# Autodesk Inventor assembly: cosel-psu-din-clip
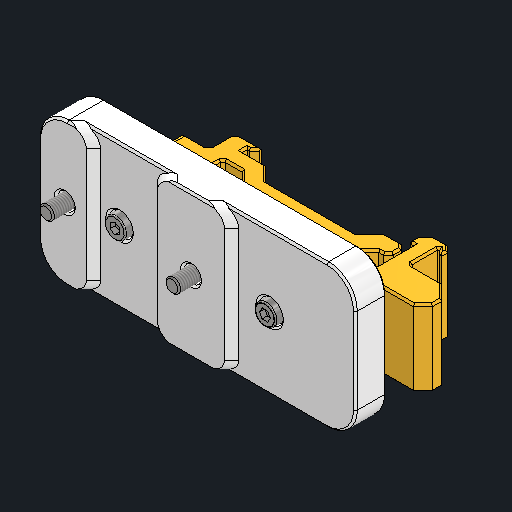
[picture p0: Inventor's stored thumbnail of the model, 512x512]
Saved by Autodesk Inventor 2026 (Build 300175050, 175E)
## iProperties
Created: 2026-03-04
Part Number: cosel-psu-din-clip
Document SubType Name: Assembly
Designer: kuzmin
Author: kuzmin
## Documents named in this file (5)
- C:\Users\queez\Dropbox\Drawings\PIHTI\ElectronicsBox\Win-GPIO-Box\cosel-psu-din-clip.iam
- C:\Users\queez\Dropbox\Drawings\PIHTI\ElectronicsBox\Win-GPIO-Box\Wide Din Clip.ipt
- C:\Users\queez\Dropbox\Drawings\PIHTI\ElectronicsBox\Win-GPIO-Box\cosel-psu-bracket.ipt
- C:\Users\queez\Dropbox\Drawings\PIHTI\ContentCenter\Fastners\M2.5x10-SHCS.ipt
- C:\Users\queez\Dropbox\Drawings\PIHTI\ContentCenter\Fastners\M3x12-SHCS.ipt
## Components (6 placed, 4 different names)
1. Wide Din Clip:1
2. cosel-psu-bracket:1 — Rigid:2, Rigid:3, Mate:1, Mate:2, Rigid:4
3. BS EN ISO 4762 - Metric M2,5 x 10:1 — Rigid:2
4. BS EN ISO 4762 - Metric M2,5 x 10:2 — Rigid:3
5. AS 1420 - Metric M3 x 12:1 — Mate:1, Mate:2
6. AS 1420 - Metric M3 x 12:2 — Rigid:4
## Relationships (5: WeldJoint 3, Mate 2)
- Rigid:2 [WeldJoint]: cosel-psu-bracket:1 ↔ BS EN ISO 4762 - Metric M2,5 x 10:1
- Rigid:3 [WeldJoint]: cosel-psu-bracket:1 ↔ BS EN ISO 4762 - Metric M2,5 x 10:2
- Mate:1: cosel-psu-bracket:1 ↔ AS 1420 - Metric M3 x 12:1
- Mate:2: cosel-psu-bracket:1 ↔ AS 1420 - Metric M3 x 12:1
- Rigid:4 [WeldJoint]: cosel-psu-bracket:1 ↔ AS 1420 - Metric M3 x 12:2
